# Autodesk Inventor assembly: Montagizinha
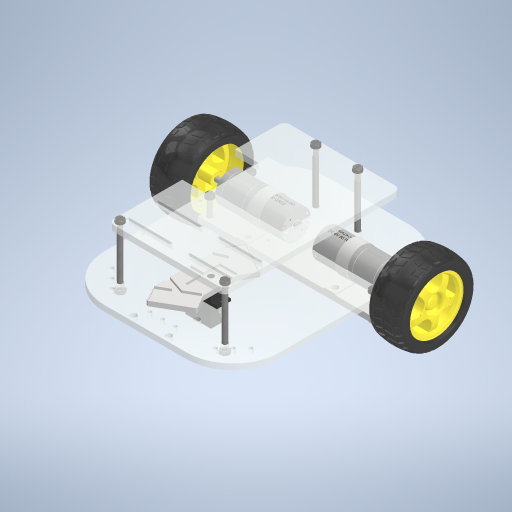
[picture p0: Inventor's stored thumbnail of the model, 512x512]
Saved by Autodesk Inventor 2024 (Build 280153020, 153B)
## iProperties
Created: 2023-06-05
Part Number: Montagizinha
Document SubType Name: Assembly
Designer: victo
Author: victo
## Documents named in this file (15)
- C:\Users\victo\Área de Trabalho\Escola\Estágio CEFET\Projeto Lidar\Projeto\Peças\Montagizinha.iam
- C:\Users\victo\Área de Trabalho\Escola\Estágio CEFET\Projeto Lidar\Projeto\Peças\BaseP.ipt
- C:\Users\victo\OneDrive\Documentos\Inventor\Content Center Files\R2024\pt-BR\AS 1474(1)\AS 1474 - M4(1).ipt
- C:\Users\victo\Área de Trabalho\Escola\Estágio CEFET\Projeto Lidar\Projeto\Peças\servo motor (mg90s) .ipt
- C:\Users\victo\Área de Trabalho\Escola\Estágio CEFET\Projeto Lidar\Projeto\Peças\Suporte.ipt
- C:\Users\victo\Área de Trabalho\Escola\Estágio CEFET\Projeto Lidar\Projeto\Peças\BaseS.ipt
- C:\Users\victo\OneDrive\Documentos\Inventor\Content Center Files\R2024\pt-BR\CSN 02 1131  B\CSN 02 1131 - M4 x 45B.ipt
- C:\Users\victo\OneDrive\Documentos\Inventor\Content Center Files\R2024\pt-BR\CSN 02 1131  B\CSN 02 1131 - M1,6 x 10B.ipt
- C:\Users\victo\OneDrive\Documentos\Inventor\Content Center Files\R2024\pt-BR\AS 1474(1)\AS 1474 - M1,6(1).ipt
- C:\Users\victo\Área de Trabalho\Escola\Estágio CEFET\Projeto Lidar\Projeto\Peças\apoiom.ipt
- C:\Users\victo\Área de Trabalho\Escola\Estágio CEFET\Projeto Lidar\Projeto\Peças\BaseM.ipt
- C:\Users\victo\OneDrive\Documentos\Inventor\Content Center Files\R2024\pt-BR\CSN 02 1131  B\CSN 02 1131 - M4 x 14B.ipt
- C:\Users\victo\OneDrive\Documentos\Inventor\Content Center Files\R2024\pt-BR\CSN 02 1131  B\CSN 02 1131 - M4 x 10B.ipt
- C:\Users\victo\Área de Trabalho\Escola\Estágio CEFET\Projeto Lidar\Projeto\Peças\motorreductor v4\motorreductor v4.ipt
- C:\Users\victo\Área de Trabalho\Escola\Estágio CEFET\Projeto Lidar\Projeto\Peças\wheel (scaled)\wheel (scaled).ipt
## Components (29 placed, 14 different names)
1. BaseP:1 — Coincidente:18, Coincidente:20, Coincidente:22, Coincidente:23, Coincidente:25, Inserir:1, Inserir:2, Coincidente:26, Coincidente:28, Coincidente:36, Coincidente:38, Inserir:7, Inserir:8, Inserir:9, Inserir:10
2. servo motor (mg90s) :1 — Coincidente:18, Coincidente:20, Coincidente:22, Coincidente:23, Coincidente:24, Coincidente:25
3. Suporte:1 — Coincidente:24
4. CSN 02 1131 B M1,6 x 10:1 — Inserir:1, Coincidente:35
5. CSN 02 1131 B M1,6 x 10:2 — Inserir:2, Coincidente:37
6. BaseS:1 — Inserir:3, Inserir:4, Inserir:5, Inserir:6, Coincidente:27
7. CSN 02 1131 B M4 x 45:1 — Inserir:3, Coincidente:26
8. CSN 02 1131 B M4 x 45:2 — Inserir:4
9. CSN 02 1131 B M4 x 45:3 — Inserir:5, Coincidente:34
10. CSN 02 1131 B M4 x 45:4 — Inserir:6, Coincidente:27, Coincidente:28, Coincidente:33
11. AS 1474 - Métrica M4:7 — Coincidente:33
12. AS 1474 - Métrica M4:8 — Coincidente:34
13. AS 1474 - Métrica M1,6:1 — Coincidente:35, Coincidente:36
14. AS 1474 - Métrica M1,6:2 — Coincidente:37, Coincidente:38
15. apoiom:1 — Coincidente:48, Coincidente:50
16. apoiom:2 — Coincidente:49, Coincidente:52
17. CSN 02 1131 B M4 x 14:4 — Inserir:7
18. CSN 02 1131 B M4 x 14:1 — Inserir:8, Coincidente:39
19. CSN 02 1131 B M4 x 14:2 — Inserir:9
20. CSN 02 1131 B M4 x 14:3 — Inserir:10
21. BaseM:1 — Coincidente:39, Coincidente:40, Coincidente:41, Coincidente:42, Coincidente:43, Coincidente:44, Coincidente:45, Coincidente:46, Coincidente:47, Coincidente:48, Coincidente:49
22. CSN 02 1131 B M4 x 10:1 — Coincidente:40, Coincidente:41
23. CSN 02 1131 B M4 x 10:2 — Coincidente:42, Coincidente:43
24. CSN 02 1131 B M4 x 10:3 — Coincidente:44, Coincidente:45
25. CSN 02 1131 B M4 x 10:4 — Coincidente:46, Coincidente:47
26. motorreductor v4:1 — Coincidente:50, Coincidente:51
27. motorreductor v4:2 — Coincidente:52, Coincidente:53
28. wheel (scaled):1 — Coincidente:53
29. wheel (scaled):3 — Coincidente:51
## Relationships (40: Mate 30, Insert 10)
- Coincidente:18 [Mate]: BaseP:1 ↔ servo motor (mg90s) :1
- Coincidente:20 [Mate]: BaseP:1 ↔ servo motor (mg90s) :1
- Coincidente:22 [Mate]: BaseP:1 ↔ servo motor (mg90s) :1
- Coincidente:23 [Mate]: BaseP:1 ↔ servo motor (mg90s) :1
- Coincidente:24 [Mate]: servo motor (mg90s) :1 ↔ Suporte:1
- Coincidente:25 [Mate]: BaseP:1 ↔ servo motor (mg90s) :1
- Inserir:1: BaseP:1 ↔ CSN 02 1131 B M1,6 x 10:1
- Inserir:2: BaseP:1 ↔ CSN 02 1131 B M1,6 x 10:2
- Inserir:3: BaseS:1 ↔ CSN 02 1131 B M4 x 45:1
- Inserir:4: BaseS:1 ↔ CSN 02 1131 B M4 x 45:2
- Inserir:5: BaseS:1 ↔ CSN 02 1131 B M4 x 45:3
- Inserir:6: BaseS:1 ↔ CSN 02 1131 B M4 x 45:4
- Coincidente:26 [Mate]: BaseP:1 ↔ CSN 02 1131 B M4 x 45:1
- Coincidente:27 [Mate]: BaseS:1 ↔ CSN 02 1131 B M4 x 45:4
- Coincidente:28 [Mate]: BaseP:1 ↔ CSN 02 1131 B M4 x 45:4
- Coincidente:33 [Mate]: CSN 02 1131 B M4 x 45:4 ↔ AS 1474 - Métrica M4:7
- Coincidente:34 [Mate]: CSN 02 1131 B M4 x 45:3 ↔ AS 1474 - Métrica M4:8
- Coincidente:35 [Mate]: CSN 02 1131 B M1,6 x 10:1 ↔ AS 1474 - Métrica M1,6:1
- Coincidente:36 [Mate]: BaseP:1 ↔ AS 1474 - Métrica M1,6:1
- Coincidente:37 [Mate]: CSN 02 1131 B M1,6 x 10:2 ↔ AS 1474 - Métrica M1,6:2
- Coincidente:38 [Mate]: BaseP:1 ↔ AS 1474 - Métrica M1,6:2
- Inserir:7: BaseP:1 ↔ CSN 02 1131 B M4 x 14:4
- Inserir:8: BaseP:1 ↔ CSN 02 1131 B M4 x 14:1
- Inserir:9: BaseP:1 ↔ CSN 02 1131 B M4 x 14:2
- Inserir:10: BaseP:1 ↔ CSN 02 1131 B M4 x 14:3
- Coincidente:39 [Mate]: CSN 02 1131 B M4 x 14:1 ↔ BaseM:1
- Coincidente:40 [Mate]: BaseM:1 ↔ CSN 02 1131 B M4 x 10:1
- Coincidente:41 [Mate]: BaseM:1 ↔ CSN 02 1131 B M4 x 10:1
- Coincidente:42 [Mate]: BaseM:1 ↔ CSN 02 1131 B M4 x 10:2
- Coincidente:43 [Mate]: BaseM:1 ↔ CSN 02 1131 B M4 x 10:2
- Coincidente:44 [Mate]: BaseM:1 ↔ CSN 02 1131 B M4 x 10:3
- Coincidente:45 [Mate]: BaseM:1 ↔ CSN 02 1131 B M4 x 10:3
- Coincidente:46 [Mate]: BaseM:1 ↔ CSN 02 1131 B M4 x 10:4
- Coincidente:47 [Mate]: BaseM:1 ↔ CSN 02 1131 B M4 x 10:4
- Coincidente:48 [Mate]: apoiom:1 ↔ BaseM:1
- Coincidente:49 [Mate]: apoiom:2 ↔ BaseM:1
- Coincidente:50 [Mate]: apoiom:1 ↔ motorreductor v4:1
- Coincidente:51 [Mate]: motorreductor v4:1 ↔ wheel (scaled):3
- Coincidente:52 [Mate]: apoiom:2 ↔ motorreductor v4:2
- Coincidente:53 [Mate]: motorreductor v4:2 ↔ wheel (scaled):1
